# Autodesk Inventor assembly: Spinn105_Subrack
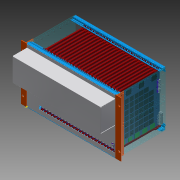
[picture p0: Inventor's stored thumbnail of the model, 180x180]
Saved by Autodesk Inventor 2015 SP1 (Build 190203100, 203)
## iProperties
Created: 2014-08-23
Part Number: Spinn105_Subrack
Document SubType Name: Assembly
Designer: Patrick Camilleri
Author: Patrick Camilleri
## Documents named in this file (6)
- C:\Users\Patrick\CAD\Spin5 Subrack\Spinn105_Subrack.iam
- C:\Users\Patrick\CAD\Spin5 Subrack\GuideRail_24560353.ipt
- C:\Users\Patrick\CAD\Spin5 Subrack\Imported Components\24563492\24563492.iam
- C:\Users\Patrick\CAD\Spin5 Board\Spin5 Inventor Simple 2\Imported Components\spin5v1_simple_2\spin5v1_simple_2.iam
- C:\Users\Patrick\CAD\Spin5 Subrack\subrack_frontpanel.ipt
- C:\Users\Patrick\CAD\Sata Shielding\Shield.ipt
## Components (75 placed, 5 different names)
1. 24563492:1 [sub-assembly] — Rigid:3, Rigid:4, Mate:1, Mate:2
2. subrack_frontpanel:1 — Mate:4, Rigid:6
3. Shield:1 — Rigid:6
4. GuideRail_24560353:1 — Rigid:3, Rigid:5
5. GuideRail_24560353:3
6. GuideRail_24560353:4
7. GuideRail_24560353:5
8. GuideRail_24560353:6
9. GuideRail_24560353:7
10. GuideRail_24560353:8
11. GuideRail_24560353:9
12. GuideRail_24560353:10
13. GuideRail_24560353:11
14. GuideRail_24560353:12
15. GuideRail_24560353:13
16. GuideRail_24560353:14
17. GuideRail_24560353:15
18. GuideRail_24560353:16
19. GuideRail_24560353:17
20. GuideRail_24560353:18
21. GuideRail_24560353:19
22. GuideRail_24560353:20
23. GuideRail_24560353:21
24. GuideRail_24560353:22
25. GuideRail_24560353:23
26. GuideRail_24560353:24
27. GuideRail_24560353:25
28. GuideRail_24560353:2 — Rigid:4
29. GuideRail_24560353:26
30. GuideRail_24560353:27
31. GuideRail_24560353:28
32. GuideRail_24560353:29
33. GuideRail_24560353:30
34. GuideRail_24560353:31
35. GuideRail_24560353:32
36. GuideRail_24560353:33
37. GuideRail_24560353:34
38. GuideRail_24560353:35
39. GuideRail_24560353:36
40. GuideRail_24560353:37
41. GuideRail_24560353:38
42. GuideRail_24560353:39
43. GuideRail_24560353:40
44. GuideRail_24560353:41
45. GuideRail_24560353:42
46. GuideRail_24560353:43
47. GuideRail_24560353:44
48. GuideRail_24560353:45
49. GuideRail_24560353:46
50. GuideRail_24560353:47
51. GuideRail_24560353:48
52. spin5v1_simple_2:1 [sub-assembly] — Rigid:5
53. spin5v1_simple_2:2 [sub-assembly]
54. spin5v1_simple_2:3 [sub-assembly]
55. spin5v1_simple_2:4 [sub-assembly]
56. spin5v1_simple_2:5 [sub-assembly]
57. spin5v1_simple_2:6 [sub-assembly]
58. spin5v1_simple_2:7 [sub-assembly]
59. spin5v1_simple_2:8 [sub-assembly]
60. spin5v1_simple_2:9 [sub-assembly]
61. spin5v1_simple_2:10 [sub-assembly]
62. spin5v1_simple_2:11 [sub-assembly]
63. spin5v1_simple_2:12 [sub-assembly]
64. spin5v1_simple_2:13 [sub-assembly]
65. spin5v1_simple_2:14 [sub-assembly]
66. spin5v1_simple_2:15 [sub-assembly]
67. spin5v1_simple_2:16 [sub-assembly]
68. spin5v1_simple_2:17 [sub-assembly]
69. spin5v1_simple_2:18 [sub-assembly]
70. spin5v1_simple_2:19 [sub-assembly]
71. spin5v1_simple_2:20 [sub-assembly]
72. spin5v1_simple_2:21 [sub-assembly]
73. spin5v1_simple_2:22 [sub-assembly]
74. spin5v1_simple_2:23 [sub-assembly]
75. spin5v1_simple_2:24 [sub-assembly]
## Component patterns: (24 elements, first: GuideRail_24560353:1), (24 elements, first: GuideRail_24560353:2), (24 elements, first: spin5v1_simple_2:1)
## Relationships (8: WeldJoint 4, Mate 4)
- Rigid:3 [WeldJoint]: 24563492:1 ↔ GuideRail_24560353:1
- Rigid:4 [WeldJoint]: 24563492:1 ↔ GuideRail_24560353:2
- Mate:1: 24563492:1
- Mate:2: 24563492:1
- Mate:3
- Mate:4: subrack_frontpanel:1
- Rigid:5 [WeldJoint]: GuideRail_24560353:1 ↔ spin5v1_simple_2:1
- Rigid:6 [WeldJoint]: subrack_frontpanel:1 ↔ Shield:1
